# Autodesk Inventor assembly: NTC thermistor
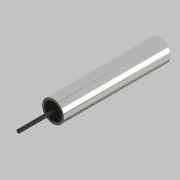
[picture p0: Inventor's stored thumbnail of the model, 180x180]
Saved by Autodesk Inventor 2020 (Build 240168000, 168)
## iProperties
Created: 2020-01-27
Part Number: NTC thermistor
Document SubType Name: Assembly
Designer: Abbas
Sending System: SolidWorks 2018
Last Author: Ingenieria_3
Last Saved: 2020-01-27
Author: Abbas
## Documents named in this file (4)
- C:\Users\LENOVO\Desktop\Graduation Project\Fish Farming Unit\Sensors\ntc-thermistor-2.snapshot.1\NTC Thermistor\NTC thermistor.iam
- C:\Users\LENOVO\Desktop\Graduation Project\Fish Farming Unit\Sensors\ntc-thermistor-2.snapshot.1\NTC Thermistor\Steel case.ipt
- C:\Users\LENOVO\Desktop\Graduation Project\Fish Farming Unit\Sensors\ntc-thermistor-2.snapshot.1\NTC Thermistor\Thermistor.ipt
- C:\Users\LENOVO\Desktop\Graduation Project\Fish Farming Unit\Sensors\ntc-thermistor-2.snapshot.1\NTC Thermistor\Cover.ipt
## Components (3 placed, 3 different names)
1. Thermistor:1
2. Cover:1 — Mate:1
3. Steel case:1 — Mate:1
## Relationships (1: Mate 1)
- Mate:1: Cover:1 ↔ Steel case:1
